# Autodesk Inventor assembly: AM Shifter Output Shaft subassembly
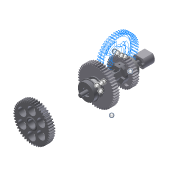
[picture p0: Inventor's stored thumbnail of the model, 180x180]
Saved by Autodesk Inventor 2013 (Build 170138000, 138)
## iProperties
Created: 2012-06-03
Part Number: AM Shifter Output Shaft subassembly
Document SubType Name: Assembly
Designer: Nemo
Mass: 414.858 g
Surface Area: 471.715 cm^2
Volume: 78.5998 cm^3
Density: 5.27811 g/cm^3
Author: Nemo
## Documents named in this file (13)
- H:\Nemo\Documents\Robotics\COTS Parts\Gearboxes\Shafts\446 Shifter Shaft.iam
- H:\Nemo\Documents\Robotics\COTS Parts\Gearboxes\Shafts\AM Shifter Output Hex Shaft.ipt
- H:\Nemo\Documents\Robotics\COTS Parts\Gearboxes\Bearings\Bearing FR8zz.ipt
- H:\Nemo\Documents\Robotics\COTS Parts\Gearboxes\Bearings\Bearing FR6.ipt
- H:\Nemo\Documents\Robotics\COTS Parts\Gearboxes\Gears\Gear 20dp 875dog 35T.ipt
- H:\Nemo\Documents\Robotics\COTS Parts\Gearboxes\Shifters\Dog Gear.ipt
- H:\Nemo\Documents\Robotics\COTS Parts\Gearboxes\Shifters\Roll Pin 925x100.ipt
- H:\Nemo\Documents\Robotics\COTS Parts\Gearboxes\Shifters\Shift Block subassembly.iam
- H:\Nemo\Documents\Robotics\COTS Parts\Gearboxes\Gears\Gear 20dp 1125dog 48T.ipt
- H:\Nemo\Documents\Robotics\COTS Parts\Gearboxes\Bearings\Bearing R8.ipt
- H:\Nemo\Documents\Robotics\COTS Parts\Gearboxes\Spacers\446 shifter shaft spacer.ipt
- H:\Nemo\Documents\Robotics\COTS Parts\Gearboxes\Gears\Gear 20dp 500key 48T.ipt
- H:\Nemo\Documents\Robotics\COTS Parts\Gearboxes\Bearings\Bearing 375 ID 1125 OD flanged.ipt
## Components (12 placed, 12 different names)
1. AM Shifter Output Hex Shaft:1 — Mate:1, Insert:4, Mate:3, Angle:1, Mate:4, Mate:9, Mate:10, Angle:2, Mate:15
2. Bearing FR8zz:1 — Mate:1, Mate:12, Mate:14
3. Bearing FR6:1 — Insert:2, Insert:4, Mate:13
4. Gear 35T dog shift:1 — Insert:2
5. Dog Gear:1 — Mate:3, Angle:1, Insert:5
6. Roll Pin 925x100:1 — Insert:5, Mate:5
7. Shift Block subassembly:1 [sub-assembly] — Mate:4, Mate:5, Mate:11
8. Gear 48T dog shift:1 — Insert:6
9. Bearing R8:1 — Insert:6, Mate:9
10. 446 shifter shaft spacer:1 — Mate:15
11. Gear 48T 20dp 500hex:1 — Mate:10, Angle:2, Mate:14
12. Bearing 375 ID 1125 OD flanged:1 — Mate:11, Mate:12, Mate:13
## Relationships (17: Mate 11, Insert 4, Angle 2)
- Mate:1: AM Shifter Output Hex Shaft:1 ↔ Bearing FR8zz:1
- Insert:2: Bearing FR6:1 ↔ Gear 35T dog shift:1
- Insert:4: AM Shifter Output Hex Shaft:1 ↔ Bearing FR6:1
- Mate:3: AM Shifter Output Hex Shaft:1 ↔ Dog Gear:1
- Angle:1 (0 deg): AM Shifter Output Hex Shaft:1 ↔ Dog Gear:1
- Insert:5: Dog Gear:1 ↔ Roll Pin 925x100:1
- Mate:4: AM Shifter Output Hex Shaft:1 ↔ Shift Block subassembly:1
- Mate:5: Roll Pin 925x100:1 ↔ Shift Block subassembly:1
- Insert:6: Gear 48T dog shift:1 ↔ Bearing R8:1
- Mate:9: AM Shifter Output Hex Shaft:1 ↔ Bearing R8:1
- Mate:10: AM Shifter Output Hex Shaft:1 ↔ Gear 48T 20dp 500hex:1
- Angle:2 (0 deg): AM Shifter Output Hex Shaft:1 ↔ Gear 48T 20dp 500hex:1
- Mate:11: Shift Block subassembly:1 ↔ Bearing 375 ID 1125 OD flanged:1
- Mate:12 (-66.04 mm): Bearing FR8zz:1 ↔ Bearing 375 ID 1125 OD flanged:1
- Mate:13: Bearing FR6:1 ↔ Bearing 375 ID 1125 OD flanged:1
- Mate:14: Bearing FR8zz:1 ↔ Gear 48T 20dp 500hex:1
- Mate:15: AM Shifter Output Hex Shaft:1 ↔ 446 shifter shaft spacer:1
